# Autodesk Inventor assembly: Banebots RS-775 P60 Planetary Gearbox 1-Stage (0.5x1.5 shaft)
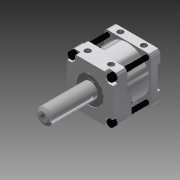
[picture p0: Inventor's stored thumbnail of the model, 180x180]
Saved by Autodesk Inventor 2014 SP1 (Build 180222100, 222)
## iProperties
Created: 2012-01-14
Part Number: Banebots RS-775 P60 Planetary Gearbox 1-Stage (0.5x1.5 shaft)
Document SubType Name: Assembly
Designer: Moses
Mass: 191.304 g
Surface Area: 316.851 cm^2
Volume: 42.8408 cm^3
Density: 4.46546 g/cm^3
Author: Moses
## Documents named in this file (12)
- C:\Users\Moses\Documents\GitHub\frc2014CAD\2012\Repackaged_Team_3061_Yr2012_Ball_Shooter\Banebots RS-775 P60 Planetary Gearbox 1-Stage (0.5x1.5 shaft).iam
- C:\Users\Moses\Documents\GitHub\frc2014CAD\2012\Repackaged_Team_3061_Yr2012_Ball_Shooter\Banebots 0.5x1.5 P60 Shaft.ipt
- C:\Users\Moses\Documents\GitHub\frc2014CAD\2012\Repackaged_Team_3061_Yr2012_Ball_Shooter\P60 Carrier Plate (output).ipt
- C:\Users\Moses\Documents\GitHub\frc2014CAD\2012\Repackaged_Team_3061_Yr2012_Ball_Shooter\15T Gear P60.ipt
- C:\Users\Moses\Documents\GitHub\frc2014CAD\2012\Repackaged_Team_3061_Yr2012_Ball_Shooter\Gearbox Pin.ipt
- C:\Users\Moses\Documents\GitHub\frc2014CAD\2012\Repackaged_Team_3061_Yr2012_Ball_Shooter\6384K540.ipt
- C:\Users\Moses\Documents\GitHub\frc2014CAD\2012\Repackaged_Team_3061_Yr2012_Ball_Shooter\P60 Gearbox End Plate.ipt
- C:\Users\Moses\Documents\GitHub\frc2014CAD\2012\Repackaged_Team_3061_Yr2012_Ball_Shooter\P60 Gearbox End Plate 2.ipt
- C:\Users\Moses\Documents\GitHub\frc2014CAD\2012\Repackaged_Team_3061_Yr2012_Ball_Shooter\91251A155.ipt
- C:\Users\Moses\Documents\GitHub\frc2014CAD\2012\Repackaged_Team_3061_Yr2012_Ball_Shooter\P60 Ring Gear 1-Stage.ipt
- C:\Users\Moses\Documents\GitHub\frc2014CAD\2012\Repackaged_Team_3061_Yr2012_Ball_Shooter\97633A170.ipt
- C:\Users\Moses\Documents\GitHub\frc2014CAD\2012\Repackaged_Team_3061_Yr2012_Ball_Shooter\P60 Shaft Shim.ipt
## Components (21 placed, 11 different names)
1. P60 Gearbox End Plate:1 — Insert:2, Flush:1, Flush:2, Mate:16, Mate:17, Mate:18, Mate:19, Mate:20, Mate:21, Mate:22, Mate:23, Insert:24, Insert:25, Insert:26, Insert:27, Insert:28, Insert:29, Insert:31
2. P60 Ring Gear 1-Stage:1 — Insert:2, Insert:3, Tangent:1, Tangent:2, Tangent:3, Tangent:4
3. P60 Gearbox End Plate 2:1 — Insert:3, Flush:1, Flush:2
4. Banebots 0.5x1.5 P60 Shaft:1 — Mate:13, Mate:14, Mate:15, Insert:30, Mate:24, Mate:25, Rotation:20
5. P60 Carrier Plate (output):1 — Insert:20, Insert:21, Insert:22, Insert:23, Mate:13, Mate:14, Mate:15, Rotation:16, Rotation:17, Rotation:18, Rotation:19
6. 15T Gear P60:13 — Insert:20, Rotation:18
7. 15T Gear P60:14 — Insert:21, Rotation:19
8. 15T Gear P60:15 — Insert:22, Rotation:17
9. 15T Gear P60:16 — Insert:23, Rotation:16
10. Gearbox Pin:1 — Mate:16, Mate:22, Tangent:1
11. Gearbox Pin:2 — Mate:17, Mate:23, Tangent:2
12. Gearbox Pin:3 — Mate:18, Mate:20, Tangent:3
13. Gearbox Pin:4 — Mate:19, Mate:21, Tangent:4
14. 6384K540:1 — Insert:24, Insert:30
15. 6384K540:2 — Insert:25
16. 91251A155:1 — Insert:26
17. 91251A155:2 — Insert:27
18. 91251A155:3 — Insert:29
19. 91251A155:4 — Insert:28
20. 97633A170:1 — Mate:24, Mate:25, Rotation:20
21. P60 Shaft Shim:1 — Insert:31
## Relationships (38: Insert 14, Mate 13, RelateRotation 5, Tangent 4, Flush 2)
- Insert:2: P60 Gearbox End Plate:1 ↔ P60 Ring Gear 1-Stage:1
- Insert:3: P60 Ring Gear 1-Stage:1 ↔ P60 Gearbox End Plate 2:1
- Flush:1: P60 Gearbox End Plate:1 ↔ P60 Gearbox End Plate 2:1
- Flush:2: P60 Gearbox End Plate:1 ↔ P60 Gearbox End Plate 2:1
- Insert:20: P60 Carrier Plate (output):1 ↔ 15T Gear P60:13
- Insert:21: P60 Carrier Plate (output):1 ↔ 15T Gear P60:14
- Insert:22: P60 Carrier Plate (output):1 ↔ 15T Gear P60:15
- Insert:23: P60 Carrier Plate (output):1 ↔ 15T Gear P60:16
- Mate:13: Banebots 0.5x1.5 P60 Shaft:1 ↔ P60 Carrier Plate (output):1
- Mate:14: Banebots 0.5x1.5 P60 Shaft:1 ↔ P60 Carrier Plate (output):1
- Mate:15: Banebots 0.5x1.5 P60 Shaft:1 ↔ P60 Carrier Plate (output):1
- Mate:16: P60 Gearbox End Plate:1 ↔ Gearbox Pin:1
- Mate:17: P60 Gearbox End Plate:1 ↔ Gearbox Pin:2
- Mate:18: P60 Gearbox End Plate:1 ↔ Gearbox Pin:3
- Mate:19: P60 Gearbox End Plate:1 ↔ Gearbox Pin:4
- Mate:20: P60 Gearbox End Plate:1 ↔ Gearbox Pin:3
- Mate:21: P60 Gearbox End Plate:1 ↔ Gearbox Pin:4
- Mate:22: P60 Gearbox End Plate:1 ↔ Gearbox Pin:1
- Mate:23: P60 Gearbox End Plate:1 ↔ Gearbox Pin:2
- Tangent:1: P60 Ring Gear 1-Stage:1 ↔ Gearbox Pin:1
- Tangent:2: P60 Ring Gear 1-Stage:1 ↔ Gearbox Pin:2
- Tangent:3: P60 Ring Gear 1-Stage:1 ↔ Gearbox Pin:3
- Tangent:4: P60 Ring Gear 1-Stage:1 ↔ Gearbox Pin:4
- Insert:24: P60 Gearbox End Plate:1 ↔ 6384K540:1
- Insert:25: P60 Gearbox End Plate:1 ↔ 6384K540:2
- Insert:26: P60 Gearbox End Plate:1 ↔ 91251A155:1
- Insert:27: P60 Gearbox End Plate:1 ↔ 91251A155:2
- Insert:28: P60 Gearbox End Plate:1 ↔ 91251A155:4
- Insert:29: P60 Gearbox End Plate:1 ↔ 91251A155:3
- Insert:30: Banebots 0.5x1.5 P60 Shaft:1 ↔ 6384K540:1
- Rotation:16 [RelateRotation] (0.5 ul): P60 Carrier Plate (output):1 ↔ 15T Gear P60:16
- Rotation:17 [RelateRotation] (0.5 ul): P60 Carrier Plate (output):1 ↔ 15T Gear P60:15
- Rotation:18 [RelateRotation] (0.5 ul): P60 Carrier Plate (output):1 ↔ 15T Gear P60:13
- Rotation:19 [RelateRotation] (0.5 ul): P60 Carrier Plate (output):1 ↔ 15T Gear P60:14
- Mate:24: Banebots 0.5x1.5 P60 Shaft:1 ↔ 97633A170:1
- Mate:25: Banebots 0.5x1.5 P60 Shaft:1 ↔ 97633A170:1
- Rotation:20 [RelateRotation] (1 ul): Banebots 0.5x1.5 P60 Shaft:1 ↔ 97633A170:1
- Insert:31: P60 Gearbox End Plate:1 ↔ P60 Shaft Shim:1
